# Autodesk Inventor assembly: servo
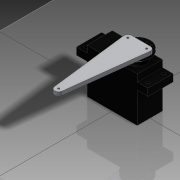
[picture p0: Inventor's stored thumbnail of the model, 180x180]
Saved by Autodesk Inventor 2013 (Build 170138000, 138)
## iProperties
Created: 2013-09-17
Part Number: servo
Document SubType Name: Assembly
Designer: Ian
Mass: 42.6263 g
Surface Area: 106.564 cm^2
Volume: 35.6368 cm^3
Density: 1.19613 g/cm^3
Author: Ian
## Documents named in this file (3)
- C:\Users\Ian\Documents\Inventor\xyPartStorage\loader\servo.iam
- C:\Users\Ian\Documents\Inventor\xyPartStorage\servo-dummy\servo-dummy.iam
- C:\Users\Ian\Documents\Inventor\xyPartStorage\loader\servo horn.ipt
## Components (2 placed, 2 different names)
1. servo-dummy:1 [sub-assembly] — Mate:1, Mate:2, Mate:3
2. servo horn:1 — Mate:1, Mate:2, Mate:3
## Relationships (3: Mate 3)
- Mate:1: servo-dummy:1 ↔ servo horn:1
- Mate:2: servo-dummy:1 ↔ servo horn:1
- Mate:3: servo-dummy:1 ↔ servo horn:1
